# Autodesk Inventor assembly: Burner_Stand_Assembly
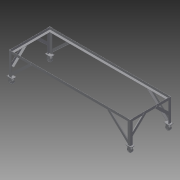
[picture p0: Inventor's stored thumbnail of the model, 180x180]
Saved by Autodesk Inventor 2014 (Build 180170000, 170)
## iProperties
Created: 2016-08-26
Part Number: Burner_Stand_Assembly
Document SubType Name: Assembly
Designer: jmw3
Author: jmw3
## Documents named in this file (4)
- F:\NIST\Project_Files\FFT_Projects\UL_Drawings\Gas_Burner\Inventor_Parts\Three_Burner_Stand_Assembly.iam
- F:\NIST\Project_Files\FFT_Projects\UL_Drawings\Gas_Burner\Inventor_Parts\Three_Burner_Stand.ipt
- F:\NIST\Project_Files\FFT_Projects\UL_Drawings\Gas_Burner\Inventor_Parts\Caster_Plate.ipt
- F:\NIST\Project_Files\FFT_Projects\UL_Drawings\Gas_Burner\Inventor_Parts\Caster.ipt
## Components (9 placed, 3 different names)
1. Three_Burner_Stand:1 — Mate:4, Flush:4, Flush:5, Mate:5, Flush:6, Flush:7, Mate:8, Flush:12, Flush:13, Mate:9, Flush:14, Flush:15
2. Caster_Plate:1 — Mate:6, Flush:8, Flush:9, Mate:9
3. Caster_Plate:2 — Mate:7, Flush:10, Flush:11, Mate:8
4. Caster_Plate:3 — Mate:1, Mate:2, Flush:1, Mate:4
5. Caster_Plate:4 — Mate:3, Flush:2, Flush:3, Mate:5
6. Caster:1 — Mate:6, Flush:8, Flush:9, Flush:14, Flush:15
7. Caster:2 — Mate:7, Flush:10, Flush:11, Flush:12, Flush:13
8. Caster:3 — Mate:3, Flush:2, Flush:3, Flush:6, Flush:7
9. Caster:4 — Mate:1, Mate:2, Flush:1, Flush:4, Flush:5
## Relationships (24: Flush 15, Mate 9)
- Mate:1: Caster_Plate:3 ↔ Caster:4
- Mate:2: Caster_Plate:3 ↔ Caster:4
- Flush:1: Caster_Plate:3 ↔ Caster:4
- Mate:3: Caster_Plate:4 ↔ Caster:3
- Flush:2: Caster_Plate:4 ↔ Caster:3
- Flush:3: Caster_Plate:4 ↔ Caster:3
- Mate:4: Three_Burner_Stand:1 ↔ Caster_Plate:3
- Flush:4 (11.1125 mm): Three_Burner_Stand:1 ↔ Caster:4
- Flush:5 (-26.9875 mm): Three_Burner_Stand:1 ↔ Caster:4
- Mate:5: Three_Burner_Stand:1 ↔ Caster_Plate:4
- Flush:6 (-26.9875 mm): Three_Burner_Stand:1 ↔ Caster:3
- Flush:7 (11.1125 mm): Three_Burner_Stand:1 ↔ Caster:3
- Mate:6: Caster_Plate:1 ↔ Caster:1
- Flush:8: Caster_Plate:1 ↔ Caster:1
- Flush:9: Caster_Plate:1 ↔ Caster:1
- Mate:7: Caster_Plate:2 ↔ Caster:2
- Flush:10: Caster_Plate:2 ↔ Caster:2
- Flush:11: Caster_Plate:2 ↔ Caster:2
- Mate:8: Three_Burner_Stand:1 ↔ Caster_Plate:2
- Flush:12 (26.9875 mm): Three_Burner_Stand:1 ↔ Caster:2
- Flush:13 (11.1125 mm): Three_Burner_Stand:1 ↔ Caster:2
- Mate:9: Three_Burner_Stand:1 ↔ Caster_Plate:1
- Flush:14 (-11.1125 mm): Three_Burner_Stand:1 ↔ Caster:1
- Flush:15 (-26.9875 mm): Three_Burner_Stand:1 ↔ Caster:1
